# Autodesk Inventor assembly: DPM_DetailedView_Assembly
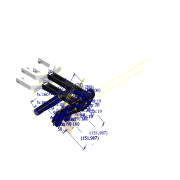
[picture p0: Inventor's stored thumbnail of the model, 180x180]
Saved by Autodesk Inventor 2022 (Build 260153000, 153)
## iProperties
Created: 2022-11-15
Part Number: DPM_DetailedView_Assembly
Document SubType Name: Assembly
Designer: alexw
Author: alexw
## Documents named in this file (8)
- C:\Users\alexw\Documents\Inventor\Projects\03_CurrentProjects\MasterThesis\PSM_V1_Rillenkugellager\DPM_DetailedView_Assembly.iam
- C:\Users\alexw\Documents\Inventor\Projects\03_CurrentProjects\MasterThesis\PSM_V1_Rillenkugellager\ParallelMechanismus_Driven_Assembly_v2.1_Rillenkugellager_Anlaufscheibe.iam
- C:\Users\alexw\Documents\Inventor\Projects\03_CurrentProjects\MasterThesis\PSM_V1_Rillenkugellager\Adaptationhorizontalachse_obereGabel_Assembly_Rillenkugellager.iam
- C:\Users\alexw\Documents\Inventor\Projects\03_CurrentProjects\MasterThesis\PSM_V1_Rillenkugellager\Adaptationhorizontalachse_Assembly_Rillenkugellager.iam
- C:\Users\alexw\Documents\Inventor\Projects\03_CurrentProjects\MasterThesis\PSM_V1_Rillenkugellager\10_79_0000_0010_003.ipt
- C:\Users\alexw\Documents\Inventor\Projects\03_CurrentProjects\MasterThesis\PSM_V1_Rillenkugellager\circlips_din471_10_1.ipt
- C:\Users\alexw\Documents\Inventor\Projects\03_CurrentProjects\MasterThesis\PSM_V1_Rillenkugellager\din_988_10_x_16_x_0_10.ipt
- C:\Users\alexw\Documents\Inventor\Projects\03_CurrentProjects\MasterThesis\PSM_V1_Rillenkugellager\ParallelMechanismus_Support_Rillenkugellager.iam
## Components (17 placed, 7 different names)
1. ParallelMechanismus_Driven_Assembly_v2.1_Rillenkugellager_Anlaufscheibe:1 [sub-assembly]
2. Adaptationhorizontalachse_obereGabel_Assembly_Rillenkugellager:1 [sub-assembly]
3. Adaptationhorizontalachse_Assembly_Rillenkugellager:1 [sub-assembly]
4. 10_79_0000_0010_003:1
5. 10_79_0000_0010_003:2
6. 10_79_0000_0010_003:3
7. 10_79_0000_0010_003:4
8. circlips_din471_10_1:1
9. circlips_din471_10_1:2
10. din_988_10_x_16_x_0_10:1
11. din_988_10_x_16_x_0_10:2
12. din_988_10_x_16_x_0_10:3
13. din_988_10_x_16_x_0_10:4
14. circlips_din471_10_1:3
15. circlips_din471_10_1:4
16. ParallelMechanismus_Support_Rillenkugellager:1 [sub-assembly]
17. ParallelMechanismus_Support_Rillenkugellager:2 [sub-assembly]
## Relationships (32: Mate 27, Flush 4, Angle 1)
- [Mate]: 10_79_0000_0010_003:1 ↔ circlips_din471_10_1:1
- [Mate]: 10_79_0000_0010_003:2 ↔ circlips_din471_10_1:2
- [Mate]: 10_79_0000_0010_003:2 ↔ din_988_10_x_16_x_0_10:1
- [Mate]: Adaptationhorizontalachse_Assembly_Rillenkugellager:1 ↔ din_988_10_x_16_x_0_10:1
- [Mate]: circlips_din471_10_1:2 ↔ din_988_10_x_16_x_0_10:1
- [Mate]: 10_79_0000_0010_003:1 ↔ din_988_10_x_16_x_0_10:2
- [Mate]: Adaptationhorizontalachse_obereGabel_Assembly_Rillenkugellager:1 ↔ din_988_10_x_16_x_0_10:2
- [Mate]: circlips_din471_10_1:1 ↔ din_988_10_x_16_x_0_10:2
- [Mate]: 10_79_0000_0010_003:3 ↔ din_988_10_x_16_x_0_10:3
- [Mate]: Adaptationhorizontalachse_Assembly_Rillenkugellager:1 ↔ din_988_10_x_16_x_0_10:3
- [Mate]: 10_79_0000_0010_003:4 ↔ din_988_10_x_16_x_0_10:4
- [Mate]: Adaptationhorizontalachse_obereGabel_Assembly_Rillenkugellager:1 ↔ din_988_10_x_16_x_0_10:4
- [Mate]: 10_79_0000_0010_003:4 ↔ circlips_din471_10_1:3
- [Mate]: din_988_10_x_16_x_0_10:4 ↔ circlips_din471_10_1:3
- [Mate]: 10_79_0000_0010_003:3 ↔ circlips_din471_10_1:4
- [Mate]: din_988_10_x_16_x_0_10:3 ↔ circlips_din471_10_1:4
- [Mate]: ParallelMechanismus_Driven_Assembly_v2.1_Rillenkugellager_Anlaufscheibe:1 ↔ Adaptationhorizontalachse_obereGabel_Assembly_Rillenkugellager:1
- [Mate]: ParallelMechanismus_Driven_Assembly_v2.1_Rillenkugellager_Anlaufscheibe:1 ↔ Adaptationhorizontalachse_Assembly_Rillenkugellager:1
- [Mate]: ParallelMechanismus_Driven_Assembly_v2.1_Rillenkugellager_Anlaufscheibe:1 ↔ Adaptationhorizontalachse_obereGabel_Assembly_Rillenkugellager:1
- [Mate]: ParallelMechanismus_Driven_Assembly_v2.1_Rillenkugellager_Anlaufscheibe:1 ↔ Adaptationhorizontalachse_Assembly_Rillenkugellager:1
- [Mate]: ParallelMechanismus_Support_Rillenkugellager:1 ↔ ParallelMechanismus_Support_Rillenkugellager:2
- [Mate]: Adaptationhorizontalachse_obereGabel_Assembly_Rillenkugellager:1 ↔ 10_79_0000_0010_003:4
- [Mate]: Adaptationhorizontalachse_Assembly_Rillenkugellager:1 ↔ 10_79_0000_0010_003:3
- [Mate]: Adaptationhorizontalachse_obereGabel_Assembly_Rillenkugellager:1 ↔ 10_79_0000_0010_003:1
- [Mate]: Adaptationhorizontalachse_Assembly_Rillenkugellager:1 ↔ 10_79_0000_0010_003:2
- [Flush]: Adaptationhorizontalachse_obereGabel_Assembly_Rillenkugellager:1 ↔ 10_79_0000_0010_003:4
- [Flush]: Adaptationhorizontalachse_Assembly_Rillenkugellager:1 ↔ 10_79_0000_0010_003:3
- [Flush]: Adaptationhorizontalachse_obereGabel_Assembly_Rillenkugellager:1 ↔ 10_79_0000_0010_003:1
- [Flush]: Adaptationhorizontalachse_Assembly_Rillenkugellager:1 ↔ 10_79_0000_0010_003:2
- [Mate]: Adaptationhorizontalachse_Assembly_Rillenkugellager:1 ↔ ParallelMechanismus_Support_Rillenkugellager:1
- [Mate]: Adaptationhorizontalachse_Assembly_Rillenkugellager:1 ↔ ParallelMechanismus_Support_Rillenkugellager:2
- [Angle] (0 deg): Adaptationhorizontalachse_obereGabel_Assembly_Rillenkugellager:1 ↔ Adaptationhorizontalachse_Assembly_Rillenkugellager:1
